# Autodesk Inventor assembly: Wheel Original_MIR
Saved by Autodesk Inventor 2014 SP1 (Build 180222100, 222)
## iProperties
Created: 2014-01-12
Part Number: Wheel Original_MIR
Document SubType Name: Assembly
Designer: tom
Author: tom
## Documents named in this file (3)
- C:\Users\tom\Documents\GitHub\Vacubot\Inventor\Wheel Original_MIR.iam
- C:\Users\tom\Documents\GitHub\Vacubot\Inventor\Wheel Bar_MIR.ipt
- C:\Users\tom\Documents\GitHub\Vacubot\Inventor\Front Wheel_MIR.ipt
## Components (2 placed, 2 different names)
1. Wheel Bar_MIR:1 — Rotational:1
2. Front Wheel_MIR:1 — Rotational:1
## Relationships (1: RevoluteJoint 1)
- Rotational:1 [RevoluteJoint]: Wheel Bar_MIR:1 ↔ Front Wheel_MIR:1
